# Autodesk Inventor assembly: Optics Assembly
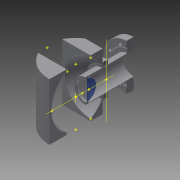
[picture p0: Inventor's stored thumbnail of the model, 180x180]
Saved by Autodesk Inventor 2015 SP1 (Build 190203100, 203)
## iProperties
Created: 2014-07-17
Part Number: Optics Assembly
Document SubType Name: Assembly
Designer: I Rabey
Author: I Rabey
## Documents named in this file (5)
- C:\ColdMatter\CADFiles\EDM Machine\Detection Region\Re-entrant Flange and Mirrors\Optics Assembly.iam
- C:\ColdMatter\CADFiles\EDM Machine\Detection Region\Re-entrant Flange and Mirrors\Mirrors\Ideas\Mirror Assembly.iam
- C:\ColdMatter\CADFiles\EDM Machine\Detection Region\Re-entrant Flange and Mirrors\Re-entrant Flange.iam
- C:\ColdMatter\CADFiles\EDM Machine\Detection Region\Re-entrant Flange and Mirrors\Mirrors\Custom Mirror Design.ipt
- C:\ColdMatter\CADFiles\EDM Machine\Detection Region\Re-entrant Flange and Mirrors\Mirrors\Custom Mirror Design Part 2.ipt
## Components (4 placed, 4 different names)
1. Mirror Assembly:1 [sub-assembly]
2. Re-entrant Flange:1 [sub-assembly] — Mate:20, Mate:21, Mate:25, Mate:28
3. Custom Mirror Design:1 — Mate:25, Mate:26
4. Custom Mirror Design Part 2:1 — Mate:21, Mate:27
## Relationships (8: Mate 8)
- Mate:11
- Mate:12
- Mate:20: Re-entrant Flange:1
- Mate:21: Re-entrant Flange:1 ↔ Custom Mirror Design Part 2:1
- Mate:25: Re-entrant Flange:1 ↔ Custom Mirror Design:1
- Mate:26 (16 mm): Custom Mirror Design:1
- Mate:27 (75 mm): Custom Mirror Design Part 2:1
- Mate:28 (32 mm): Re-entrant Flange:1
